# Autodesk Inventor assembly: Two simple doors
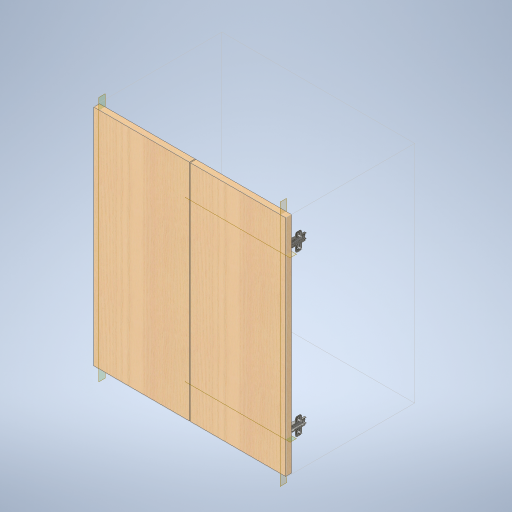
[picture p0: Inventor's stored thumbnail of the model, 512x512]
Saved by Autodesk Inventor 2024 (Build 280153000, 153)
## iProperties
Created: 2017-04-12
Part Number: Two simple doors
Document SubType Name: Assembly
Designer: SvetlanaB
Author: SvetlanaB
## Documents named in this file (7)
- C:\W4INV 2024 Design\iBOX LIBRARY\Kitchen\Doors\Two simple doors\Two simple doors.iam
- C:\W4INV 2024 Design\iBOX LIBRARY\Kitchen\Doors\Two simple doors\Right_door.ipt
- C:\W4INV 2024 Design\iBOX LIBRARY\Kitchen\Doors\Two simple doors\Left_door.ipt
- C:\W4INV 2024 Design\iBOX LIBRARY\Kitchen\Doors\Two simple doors\Two simple doors.ipt
- C:\W4INV 2024 Design\_LIBRARY\Hinges\CONCEALED HINGE\Full Overlay Hinge Wood Screw Cup Wood Screw T18.iam
- C:\W4INV 2023 Design\LIBRARY\Hinges\CONCEALED HINGE.iam
- C:\W4INV 2022 Design\iBOX LIBRARY\Kitchen\Doors\Two simple doors\Two simple doors.iam
## Components (7 placed, 4 different names)
1. Right_door:1 — Flush:1, Flush:2, Flush:3, Mate:5, Mate:7
2. Left_door:1 — Flush:4, Mate:1, Mate:3
3. @Skeleton
4. Full Overlay Hinge Wood Screw Cup Wood Screw T18:1 [sub-assembly] — Mate:1, Flush:5, Mate:2
5. Full Overlay Hinge Wood Screw Cup Wood Screw T18:2 [sub-assembly] — Mate:3, Flush:6, Mate:4
6. Full Overlay Hinge Wood Screw Cup Wood Screw T18:3 [sub-assembly] — Mate:5, Flush:7, Mate:6
7. Full Overlay Hinge Wood Screw Cup Wood Screw T18:4 [sub-assembly] — Mate:7, Flush:8, Mate:8
## Relationships (16: Flush 8, Mate 8)
- Flush:1 (-100 mm): Right_door:1
- Flush:2 (-100 mm): Right_door:1
- Flush:3 (-16.5 mm): Right_door:1
- Flush:4 (-16.5 mm): Left_door:1
- Mate:1: Left_door:1 ↔ Full Overlay Hinge Wood Screw Cup Wood Screw T18:1
- Flush:5: Full Overlay Hinge Wood Screw Cup Wood Screw T18:1
- Mate:2: Full Overlay Hinge Wood Screw Cup Wood Screw T18:1
- Mate:3: Left_door:1 ↔ Full Overlay Hinge Wood Screw Cup Wood Screw T18:2
- Flush:6: Full Overlay Hinge Wood Screw Cup Wood Screw T18:2
- Mate:4: Full Overlay Hinge Wood Screw Cup Wood Screw T18:2
- Mate:5: Right_door:1 ↔ Full Overlay Hinge Wood Screw Cup Wood Screw T18:3
- Flush:7: Full Overlay Hinge Wood Screw Cup Wood Screw T18:3
- Mate:6: Full Overlay Hinge Wood Screw Cup Wood Screw T18:3
- Mate:7: Right_door:1 ↔ Full Overlay Hinge Wood Screw Cup Wood Screw T18:4
- Flush:8: Full Overlay Hinge Wood Screw Cup Wood Screw T18:4
- Mate:8: Full Overlay Hinge Wood Screw Cup Wood Screw T18:4
## Named parameters: Width = 600 mm, Depth = 400 mm, Height = 700 mm, Top_offset = 1.5 mm, Bottom_offset = 1.5 mm, Left_offset = 1.5 mm, Right_offset = 1.5 mm, Type = 2, Panel_thickness = 18 mm, Front_offset = 2 mm, Spacing_between_doors = 3 mm, Hinge_side_offset = 18 mm, Hinge_top_offset = 100 mm, Hinge_bottom_offset = 100 mm
